# Autodesk Inventor assembly: Arm 2.0 Assembly
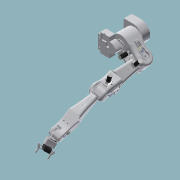
[picture p0: Inventor's stored thumbnail of the model, 180x180]
Saved by Autodesk Inventor 2017 SP1 (Build 210196100, 196)
## iProperties
Created: 2017-09-28
Part Number: Arm 2.0 Assembly
Document SubType Name: Assembly
Designer: Zach
Author: Zach
## Documents named in this file (66)
- C:\Users\Zach\Documents\GitHub\tr1\src\Body\Arm 2.0 Assembly\Arm 2.0 Assembly.iam
- C:\Users\Zach\Documents\GitHub\tr1\src\Body\Arm 2.0 Assembly\Steel Rod 8mm x 135mm.ipt
- C:\Users\Zach\Documents\GitHub\tr1\lib\22x8x8mm Bearing.ipt
- C:\Users\Zach\Documents\GitHub\tr1\src\Body\Arm 2.0 Assembly\AA004.ipt
- C:\Users\Zach\Documents\GitHub\tr1\lib\QS12MM250\QS12MM250.ipt
- C:\Users\Zach\Documents\GitHub\tr1\src\Body\Arm 2.0 Assembly\Steel Rod 8mm x 110mm.ipt
- C:\Users\Zach\Documents\GitHub\tr1\src\Body\Arm 2.0 Assembly\AA013.ipt
- C:\Users\Zach\Documents\GitHub\tr1\src\Body\Arm 2.0 Assembly\AA014.ipt
- C:\Users\Zach\Documents\GitHub\tr1\lib\12V DC Motor 378-1.ipt
- \\CR\Users\Zach\Documents\Inventor\Content Center Files\R2017\en-US\ISO 4017(1)\ISO 4017 - M5 x 20 - ISO.ipt
- C:\Users\Zach\Documents\GitHub\tr1\src\Body\Arm 2.0 Assembly\Steel Rod 8mm x 80mm.ipt
- C:\Users\Zach\Documents\GitHub\tr1\src\Body\Arm 2.0 Assembly\Gripper Assembly\Gripper B Assembly.iam
- C:\Users\Zach\Documents\GitHub\tr1\lib\8mm Hub.ipt
- C:\Users\Zach\Documents\GitHub\tr1\src\Body\Arm 2.0 Assembly\Arm 2.0 Assembly\Design Accelerator\Spur Gears5.iam
- C:\Users\Zach\Documents\GitHub\tr1\lib\4mm mounting hub.ipt
- C:\Users\Zach\Documents\GitHub\tr1\lib\6201RS\6201RS.ipt
- C:\Users\Zach\Documents\GitHub\tr1\lib\U51105\U51105.ipt
- C:\Users\Zach\Documents\GitHub\tr1\src\Body\Arm 2.0 Assembly\AA034.ipt
- C:\Users\Zach\Documents\GitHub\tr1\src\Body\Arm 2.0 Assembly\Arm 2.0 Assembly\Design Accelerator\Spur Gears6.iam
- C:\Users\Zach\Documents\GitHub\tr1\src\Body\Arm 2.0 Assembly\AA008c.ipt
- C:\Users\Zach\Documents\GitHub\tr1\src\Body\Arm 2.0 Assembly\Arm 2.0 Assembly\Design Accelerator\Spur Gears7.iam
- C:\Users\Zach\Documents\GitHub\tr1\src\Body\Arm 2.0 Assembly\AA036.ipt
- C:\Users\Zach\Documents\GitHub\tr1\src\Body\Arm 2.0 Assembly\AA037.ipt
- C:\Users\Zach\Documents\GitHub\tr1\src\Body\Arm 2.0 Assembly\AA016b.ipt
- C:\Users\Zach\Documents\GitHub\tr1\src\Body\Arm 2.0 Assembly\AA005b.ipt
- C:\Users\Zach\Documents\GitHub\tr1\src\Body\Arm 2.0 Assembly\AA006b.ipt
- C:\Users\Zach\Documents\GitHub\tr1\src\Body\Arm 2.0 Assembly\AA001c.ipt
- C:\Users\Zach\Documents\GitHub\tr1\src\Body\Arm 2.0 Assembly\Arm 2.0 Assembly\Design Accelerator\Spur Gears8.iam
- C:\Users\Zach\Documents\GitHub\tr1\src\Body\Arm 2.0 Assembly\Arm 2.0 Assembly\Design Accelerator\Spur Gears11.iam
- C:\Users\Zach\Documents\GitHub\tr1\src\Body\Arm 2.0 Assembly\Arm 2.0 Assembly\Design Accelerator\Spur Gears9.iam
- C:\Users\Zach\Documents\GitHub\tr1\src\Body\Arm 2.0 Assembly\AA010b.ipt
- C:\Users\Zach\Documents\GitHub\tr1\src\Body\Arm 2.0 Assembly\Arm 2.0 Assembly\Design Accelerator\Spur Gears10.iam
- C:\Users\Zach\Documents\GitHub\tr1\src\Body\Arm 2.0 Assembly\Arm 2.0 Assembly\Design Accelerator\Spur Gears12.iam
- C:\Users\Zach\Documents\GitHub\tr1\src\Body\Arm 2.0 Assembly\AA041.ipt
- \\CR\Users\Zach\Documents\Inventor\Content Center Files\R2017\en-US\ISO 7045  H\ISO 7045 - M3 x 8 - 4.8 - H - ISO.ipt
- C:\Users\Zach\Documents\GitHub\tr1\src\Body\Arm 2.0 Assembly\Arm 2.0 Assembly\Design Accelerator\Spur Gears13.iam
- C:\Users\Zach\Documents\GitHub\tr1\src\Body\Arm 2.0 Assembly\Arm 2.0 Assembly\Design Accelerator\Spur Gears16.iam
- C:\Users\Zach\Documents\GitHub\tr1\src\Body\Arm 2.0 Assembly\AA046.ipt
- C:\Users\Zach\Documents\GitHub\tr1\lib\MG995.ipt
- C:\Users\Zach\Documents\GitHub\tr1\lib\Servo Mounting Hub.ipt
- C:\Users\Zach\Documents\GitHub\tr1\src\Body\Arm 2.0 Assembly\AA047.ipt
- C:\Users\Zach\Documents\GitHub\tr1\src\Body\Arm 2.0 Assembly\AA048.ipt
- \\CR\Users\Zach\Documents\Inventor\Content Center Files\R2017\en-US\ISO 4018\ISO 4018 - M5 x 10.ipt
- \\CR\Users\Zach\Documents\Inventor\Content Center Files\R2017\en-US\ISO 4018\ISO 4018 - M5 x 25.ipt
- \\CR\Users\Zach\Documents\Inventor\Content Center Files\R2017\en-US\ISO 7045  H\ISO 7045 - M3 x 12 - 4.8 - H - ISO.ipt
- C:\Users\Zach\Documents\GitHub\tr1\src\Body\Arm 2.0 Assembly\AA049.ipt
- \\CR\Users\Zach\Documents\Inventor\Content Center Files\R2017\en-US\ISO 4018\ISO 4018 - M5 x 40.ipt
- \\CR\Users\Zach\Documents\Inventor\Content Center Files\R2017\en-US\ISO 4035(2)\ISO 4035 - M5 - ISO.ipt
- \\CR\Users\Zach\Documents\Inventor\Content Center Files\R2017\en-US\ISO 4018\ISO 4018 - M5 x 35.ipt
- \\CR\Users\Zach\Documents\Inventor\Content Center Files\R2017\en-US\ISO 4762(2)\ISO 4762 - M4 x 10ISO.ipt
- C:\Users\Zach\Documents\GitHub\tr1\lib\6mm Mounting Hub.ipt
- C:\Users\Zach\Documents\GitHub\tr1\src\Body\Arm 2.0 Assembly\AA035c.ipt
- C:\Users\Zach\Documents\GitHub\tr1\src\Body\Arm 2.0 Assembly\AA008d2.ipt
- C:\Users\Zach\Documents\GitHub\tr1\lib\TSINY TS-42GZ495.ipt
- C:\Users\Zach\Documents\GitHub\tr1\lib\EMS22XXX-D28-LSX.ipt
- C:\Users\Zach\Documents\GitHub\tr1\src\Body\Arm 2.0 Assembly\AA051.ipt
- C:\Users\Zach\Documents\GitHub\tr1\src\Body\Arm 2.0 Assembly\AA052.ipt
- C:\Users\Zach\Documents\GitHub\tr1\src\Body\Arm 2.0 Assembly\AA045b.ipt
- C:\Users\Zach\Documents\GitHub\tr1\lib\6mm x 120mm D Shaft.ipt
- C:\Users\Zach\Documents\GitHub\tr1\src\Body\Arm 2.0 Assembly\AA053.ipt
- C:\Users\Zach\Documents\GitHub\tr1\src\Body\Arm 2.0 Assembly\AA054.ipt
- C:\Users\Zach\Documents\GitHub\tr1\src\Body\Arm 2.0 Assembly\AA055.ipt
- \\CR\Users\Zach\Documents\Inventor\Content Center Files\R2017\en-US\AS 1421(4)\AS 1421 - M4 x 10 Flat Point.ipt
- C:\Users\Zach\Documents\GitHub\tr1\src\Body\Arm 2.0 Assembly\AA057.ipt
- C:\Users\Zach\Documents\GitHub\tr1\lib\6mm Mounting Hub, thin.ipt
- C:\Users\Zach\Documents\GitHub\tr1\lib\8mm Mounting Hub, thin.ipt
## Components (202 placed, 65 different names)
1. AA001c:1 — Mate:560, Mate:562, Mate:563, Mate:564, Mate:565, Mate:566, Mate:567, Mate:576, Mate:578, Mate:581, Mate:602, Mate:905, Mate:906, Mate:1083, Mate:1084, Mate:1085, Mate:1086, Mate:1093, Angle:18, Mate:1095, Mate:1122, Mate:1261, Mate:1262, Mate:1263, Mate:1278, Mate:1279, Mate:1280, Mate:1294
2. AA004:1 — Mate:23, Mate:345, Mate:347, Mate:350, Mate:357, Mate:590, Mate:1278
3. AA005b:1 — Mate:537, Mate:538, Mate:539, Mate:541, Mate:542, Mate:543, Mate:806, Mate:807, Mate:808, Mate:809, Mate:838, Mate:909, Mate:910
4. AA006b:1 — Mate:594, Mate:598, Mate:599, Mate:609, Mate:802, Mate:803, Mate:804, Mate:805, Mate:838, Mate:1088, Mate:1089, Angle:17, Mate:1233
5. AA008c:1 — Mate:616, Mate:1113, Mate:1114, Mate:1115, Mate:1125
6. AA008d2:1 — Mate:1104, Mate:1106, Mate:1107, Angle:22, Mate:1113, Mate:1114, Mate:1115, Mate:1124, Mate:1125, Mate:1157, Mate:1158, Mate:1159, Mate:1160, Mate:1161, Mate:1162, Mate:1163, Mate:1164, Mate:1165, Mate:1166, Mate:1170, Mate:1192, Mate:1193, Mate:1194, Mate:1195, Mate:1312
7. AA010b:1 — Mate:616, Mate:620, Mate:621, Mate:624, Mate:625, Mate:626, Mate:628, Mate:630, Mate:642, Flush:20, Mate:648, Mate:650, Mate:948, Mate:1097, Mate:1098, Angle:21, Mate:1100, Mate:1101, Mate:1102, Mate:1126, Mate:1204, Mate:1258, Mate:1259, Mate:1260, Mate:1274, Mate:1276, Mate:1277, Mate:1301
8. AA013:2 — Mate:142, Mate:143, Mate:144, Mate:145, Mate:146, Mate:147, Mate:563, Mate:564, Mate:565, Mate:1281
9. AA014:2 — Mate:628, Mate:629, Mate:630, Mate:976, Mate:977, Mate:978, Mate:979, Mate:980, Mate:981
10. AA016b:1 — Mate:518, Mate:519, Mate:520, Mate:529, Mate:530, Mate:664, Mate:665, Mate:671, Mate:673, Mate:675, Mate:676, Mate:677, Mate:877, Mate:878, Mate:1206, Mate:1207, Angle:26
11. AA034:1 — Mate:529, Mate:534, Mate:535, Mate:879, Mate:880, Mate:881, Mate:882, Mate:883, Mate:884, Mate:885, Mate:886, Mate:964, Mate:965, Mate:966, Mate:967, Mate:968, Mate:969, Mate:970, Mate:971, Mate:972, Mate:973, Mate:974, Mate:975, Mate:1213, Mate:1256, Mate:1309, Mate:1310, Mate:1311
12. AA035c:1 — Mate:1076, Mate:1077, Mate:1167, Mate:1168, Mate:1169, Mate:1170, Mate:1171, Mate:1172, Mate:1173, Mate:1175, Angle:24, Angle:25, Mate:1176, Mate:1202, Mate:1203, Angle:1297, Mate:1312
13. AA036:1 — Mate:498, Mate:501, Mate:502, Mate:511, Mate:698, Mate:868, Mate:871, Mate:872, Mate:939, Mate:1197, Mate:1198, Mate:1199, Mate:1200
14. AA037:1 — Mate:501, Mate:502, Mate:514, Mate:515, Mate:516, Mate:518, Mate:519, Mate:520, Mate:530, Mate:664, Mate:665, Mate:698, Mate:866, Mate:867, Mate:873, Mate:874, Mate:875, Mate:876, Flush:25, Flush:26, Mate:950, Mate:951, Mate:952, Mate:953
15. AA041:1 — Mate:675, Mate:676, Mate:677, Mate:682, Mate:683, Mate:684, Mate:685
16. AA045b:1 — Mate:1211, Mate:1212, Angle:27, Mate:1213, Mate:1214, Mate:1215, Mate:1216, Mate:1217, Mate:1218, Mate:1219, Flush:37, Mate:1221, Mate:1223, Mate:1224, Mate:1225, Mate:1227, Mate:1235, Mate:1264, Mate:1265, Mate:1310, Mate:1311
17. AA046:1 — Mate:727, Mate:728, Mate:731, Mate:735, Mate:736, Mate:737, Mate:752, Mate:756, Mate:758, Mate:759, Mate:760, Mate:761, Mate:762, Mate:763, Mate:1217, Mate:1296, Mate:1297
18. AA047:1 — Mate:735, Mate:736, Mate:737, Mate:738, Mate:739, Mate:740, Mate:753, Mate:754, Mate:755, Mate:800, Mate:801
19. AA048:1 — Mate:744, Mate:745, Mate:746, Mate:747, Mate:748, Mate:749
20. AA049:1 — Mate:783, Mate:786, Mate:787, Mate:788, Mate:789, Mate:790, Mate:791, Mate:1218
21. AA051:1 — Mate:1196, Mate:1197
22. AA052:1 — Mate:1201, Mate:1202
23. AA053:1 — Mate:1258, Mate:1259, Mate:1260
24. AA053:3 — Mate:1261, Mate:1262, Mate:1263
25. AA054:1 — Mate:1270, Mate:1271, Mate:1275, Mate:1276, Mate:1282, Mate:1320
26. AA055:1 — Mate:1274, Mate:1275, Mate:1277
27. AA057:1 — Mate:1293, Angle:1295, Mate:1294, Mate:1295
28. AA057:2 — Mate:1300, Angle:1296, Mate:1301, Mate:1302
29. Gripper B Assembly:1 [sub-assembly] — Mate:747, Mate:748, Mate:749
30. 22x8x8mm Bearing:1 — Mate:433, Mate:560
31. 22x8x8mm Bearing:2 — Mate:437, Mate:562
32. 22x8x8mm Bearing:3 — Mate:57, Mate:620, Mate:626
33. 22x8x8mm Bearing:4 — Mate:621, Mate:629, Mate:642
34. 22x8x8mm Bearing:5 — Mate:186, Mate:1265
35. 22x8x8mm Bearing:6 — Mate:187, Mate:1264
36. 22x8x8mm Bearing:7 — Mate:1308
37. QS12MM250:1 — Mate:23, Mate:344, Mate:346, Mate:348, Mate:354, Mate:537, Mate:594, Mate:597, Mate:1230
38. Steel Rod 8mm x 140mm:1 — Mate:433, Mate:437, Mate:476, Mate:575, Mate:651, Mate:1076, Mate:1122, Flush:35, Mate:1201
39. Steel Rod 8mm x 110mm:1 — Mate:57, Mate:491, Mate:498, Flush:20, Mate:649, Mate:1196, Mate:1204, Mate:1283
40. Steel Rod 8mm x 80mm:1 — Mate:186, Mate:187, Mate:710, Mate:721, Mate:724, Mate:730, Mate:783, Mate:1216, Flush:37, Mate:1234, Mate:1298, Mate:1299
41. TSINY TS-42GZ495:3 — Mate:1104, Mate:1160, Mate:1161, Mate:1270, Mate:1271, Angle:1297
42. TSINY TS-42GZ495:2 — Mate:1097, Mate:1098, Mate:1101, Mate:1102, Mate:1128, Mate:1300, Angle:1296
43. TSINY TS-42GZ495:1 — Mate:1083, Mate:1084, Mate:1085, Mate:1086, Mate:1293, Angle:1295
44. 12V DC Motor 378-1:3 — Mate:712, Mate:714, Mate:778, Mate:779, Mate:1224, Mate:1225
45. 12V DC Motor 378-1:4 — Mate:514, Mate:515, Mate:516, Mate:1290, Mate:1292, Mate:1303, Mate:1304
46. 12V DC Motor 378-1:6 — Mate:340, Mate:342, Mate:538, Mate:539, Mate:540, Mate:543, Mate:907, Mate:908
47. 6201RS:1 — Mate:346, Mate:347
48. 6201RS:2 — Mate:357, Mate:597
49. U51105:1 — Mate:348, Mate:349, Mate:542
50. U51105:2 — Mate:354, Mate:608, Mate:609, Mate:600
51. 6mm Mounting Hub:7 — Mate:1185, Mate:1186, Mate:1188
52. 6mm Mounting Hub:5 — Mate:1177, Mate:1178, Mate:1179
53. 6mm Mounting Hub:2 — Mate:1090, Mate:1091
54. 6mm Mounting Hub:11 — Mate:1283, Mate:1284
55. 6mm Mounting Hub:10 — Mate:1228, Mate:1323
56. 8mm Hub:2 — Mate:534, Mate:535, Mate:1306
57. 8mm Hub:4 — Mate:580, Mate:581, Mate:582, Flush:35
58. 8mm Hub:6 — Mate:651, Mate:911, Mate:912, Mate:913, Mate:914, Mate:915, Mate:916, Mate:1203
59. 8mm Hub:8 — Mate:721, Mate:1234, Mate:1324, Mate:1325
60. 8mm Hub:9 — Mate:727, Mate:728, Mate:730, Mate:756, Mate:764, Mate:765, Mate:766, Mate:767, Mate:768, Mate:769, Mate:1298, Mate:1299
61. 8mm Hub:14 — Mate:1198, Mate:1199, Mate:1200
62. 4mm mounting hub:1 — Mate:340, Mate:540, Mate:541, Mate:887
63. 4mm mounting hub:8 — Mate:714, Mate:716, Mate:782, Mate:1226
64. Servo Mounting Hub:1 — Mate:733, Mate:734, Mate:738, Mate:739, Mate:740, Mate:792, Mate:793, Mate:794, Mate:795, Mate:796, Mate:797, Mate:798, Mate:799
65. 6mm x 120mm D Shaft:1 — Mate:1292, Mate:1303, Mate:1304, Mate:1305, Mate:1306, Mate:1308, Mate:1309, Mate:1318
66. EMS22XXX-D28-LSX:1 — Mate:1088, Mate:1089, Angle:17, Mate:1090, Mate:1091, Mate:1182, Mate:1232
67. EMS22XXX-D28-LSX:2 — Mate:1093, Angle:18, Mate:1095, Mate:1177, Mate:1180
68. EMS22XXX-D28-LSX:3 — Angle:21, Mate:1100, Mate:1126, Mate:1185, Mate:1187
69. EMS22XXX-D28-LSX:4 — Mate:1106, Mate:1107, Angle:22, Mate:1190, Mate:1313
70. EMS22XXX-D28-LSX:5 — Mate:1206, Mate:1207, Angle:26, Mate:1210, Mate:1316, Mate:1326
71. EMS22XXX-D28-LSX:6 — Mate:1211, Mate:1212, Angle:27, Mate:1228, Mate:1267
72. AASG01 [sub-assembly] — Mate:342, Mate:344, Mate:345, Mate:349, Mate:350, Mate:810, Mate:811, Mate:812, Mate:813, Mate:814, Mate:815, Mate:816, Mate:817, Mate:818, Mate:819, Mate:820, Mate:821, Mate:887, Mate:888, Mate:889, Mate:890, Mate:891, Mate:1279, Mate:1280
73. AASG02 [sub-assembly] — Mate:476, Mate:566, Mate:567, Mate:602, Mate:839, Mate:841, Mate:842, Mate:843, Mate:844, Mate:845, Mate:897, Mate:898, Mate:899, Mate:900, Mate:901, Mate:902, Mate:1077, Mate:1295
74. AASG03 [sub-assembly] — Mate:491, Mate:511, Mate:624, Mate:625, Mate:860, Mate:861, Mate:862, Mate:863, Mate:864, Mate:865, Mate:1128, Mate:1302
75. AASG04 [sub-assembly] — Mate:575, Mate:576, Mate:578, Mate:580, Mate:582, Mate:917, Mate:918, Mate:919, Mate:920, Mate:921, Mate:922, Mate:1178, Mate:1179, Mate:1180
76. AASG05 [sub-assembly] — Mate:590, Mate:608, Mate:827, Mate:828, Mate:829, Mate:830, Mate:831, Mate:832, Mate:833, Mate:1182, Mate:1230, Mate:1232, Mate:1233
77. AASG06 [sub-assembly] — Mate:1124, Mate:1190, Mate:1268, Mate:1269, Mate:1282, Mate:1314, Mate:1315, Mate:1321, Mate:1322
78. AASG07 [sub-assembly] — Mate:648, Mate:649, Mate:650, Mate:958, Mate:959, Mate:960, Mate:961, Mate:962, Mate:963, Mate:1186, Mate:1187, Mate:1188, Mate:1284
79. AASG08 [sub-assembly] — Mate:671, Mate:673, Mate:680, Mate:681, Mate:1305, Mate:1317, Mate:1319, Mate:1326
80. AASG09 [sub-assembly] — Mate:710, Mate:712, Mate:716, Mate:731, Mate:770, Mate:771, Mate:772, Mate:773, Mate:774, Mate:775, Mate:776, Mate:777, Mate:782, Mate:1223, Mate:1226, Mate:1227, Mate:1296, Mate:1297
81. AASG10 [sub-assembly] — Mate:724, Mate:1221, Mate:1235, Mate:1267, Mate:1323, Mate:1324, Mate:1325
82. MG995:1 — Mate:733, Mate:734, Mate:744, Mate:745, Mate:746
83. 6mm Mounting Hub, thin:1 — Mate:1313, Mate:1314, Mate:1315
84. ISO 7045 H M3 x 8 - 4.8 - H:1 — Mate:680, Mate:681
85. ISO 7045 H M3 x 8 - 4.8 - H:2 — Mate:682, Mate:685
86. ISO 7045 H M3 x 8 - 4.8 - H:3 — Mate:683, Mate:684
87. ISO 7045 H M3 x 8 - 4.8 - H:5 — Mate:778
88. ISO 7045 H M3 x 8 - 4.8 - H:6 — Mate:779
89. ISO 7045 H M3 x 8 - 4.8 - H:7 — Mate:795, Mate:799
90. ISO 7045 H M3 x 8 - 4.8 - H:8 — Mate:794, Mate:798
91. ISO 7045 H M3 x 8 - 4.8 - H:9 — Mate:792, Mate:796
92. ISO 7045 H M3 x 8 - 4.8 - H:10 — Mate:793, Mate:797
93. ISO 7045 H M3 x 8 - 4.8 - H:11 — Mate:800, Mate:801
94. ISO 7045 H M3 x 8 - 4.8 - H:13 — Mate:897, Mate:900
95. ISO 7045 H M3 x 8 - 4.8 - H:14 — Mate:898, Mate:901
96. ISO 7045 H M3 x 8 - 4.8 - H:15 — Mate:899, Mate:902
97. ISO 7045 H M3 x 8 - 4.8 - H:16 — Mate:908, Mate:910
98. ISO 7045 H M3 x 8 - 4.8 - H:17 — Mate:907, Mate:909
99. ISO 7045 H M3 x 8 - 4.8 - H:20 — Mate:951, Mate:953
100. ISO 7045 H M3 x 8 - 4.8 - H:21 — Mate:950, Mate:952
101. ISO 7045 H M3 x 8 - 4.8 - H:24 — Mate:960, Mate:963
102. ISO 7045 H M3 x 8 - 4.8 - H:25 — Mate:958, Mate:962
103. ISO 7045 H M3 x 8 - 4.8 - H:26 — Mate:959, Mate:961
104. ISO 7045 H M3 x 8 - 4.8 - H:27 — Mate:965, Mate:972
105. ISO 7045 H M3 x 8 - 4.8 - H:28 — Mate:964, Mate:973
106. ISO 7045 H M3 x 8 - 4.8 - H:29 — Mate:966, Mate:971
107. ISO 7045 H M3 x 8 - 4.8 - H:30 — Mate:967, Mate:970, Mate:1256
108. ISO 7045 H M3 x 8 - 4.8 - H:31 — Mate:969, Mate:975
109. ISO 7045 H M3 x 8 - 4.8 - H:32 — Mate:968, Mate:974
110. ISO 7045 H M3 x 12 - 4.8 - H:1 — Mate:765, Mate:767
111. ISO 7045 H M3 x 12 - 4.8 - H:3 — Mate:764, Mate:769
112. ISO 7045 H M3 x 12 - 4.8 - H:2 — Mate:766, Mate:768
113. ISO 7045 H M3 x 12 - 4.8 - H:4 — Mate:770, Mate:775
114. ISO 7045 H M3 x 12 - 4.8 - H:5 — Mate:771, Mate:774
115. ISO 7045 H M3 x 12 - 4.8 - H:6 — Mate:773, Mate:777
116. ISO 7045 H M3 x 12 - 4.8 - H:7 — Mate:772, Mate:776
117. ISO 7045 H M3 x 12 - 4.8 - H:8 — Mate:889, Mate:890
118. ISO 7045 H M3 x 12 - 4.8 - H:9 — Mate:888, Mate:891
119. ISO 7045 H M3 x 12 - 4.8 - H:10 — Mate:911, Mate:914
120. ISO 7045 H M3 x 12 - 4.8 - H:11 — Mate:913, Mate:915
121. ISO 7045 H M3 x 12 - 4.8 - H:12 — Mate:912, Mate:916
122. ISO 7045 H M3 x 12 - 4.8 - H:13 — Mate:919, Mate:920
123. ISO 7045 H M3 x 12 - 4.8 - H:14 — Mate:917, Mate:921
124. ISO 7045 H M3 x 12 - 4.8 - H:15 — Mate:918, Mate:922
125. ISO 7045 H M3 x 12 - 4.8 - H:18
126. ISO 7045 H M3 x 12 - 4.8 - H:19
127. ISO 7045 H M3 x 12 - 4.8 - H:20
128. ISO 7045 H M3 x 12 - 4.8 - H:32 — Mate:1268, Mate:1269
129. ISO 4762 M4 x 10:1 — Mate:905
130. ISO 4762 M4 x 10:2 — Mate:906
131. ISO 4762 M4 x 10:4 — Mate:948
132. ISO 4035 M5:1 — Mate:1167, Mate:1168
133. ISO 4035 M5:2 — Mate:852, Mate:1176
134. ISO 4035 M5:3 — Mate:869, Mate:872
135. ISO 4035 M5:4 — Mate:870, Mate:871
136. ISO 4035 M5:5 — Mate:985
137. ISO 4035 M5:6 — Mate:984
138. ISO 4035 M5:7 — Mate:989
139. ISO 4035 M5:8 — Mate:988
140. ISO 4035 M5:9 — Mate:1174, Mate:1175, Angle:24
141. ISO 4035 M5:10 — Mate:1027, Mate:1173, Angle:25
142. ISO 4018 M5 x 10:1 — Mate:754, Mate:755
143. ISO 4018 M5 x 10:2 — Mate:752, Mate:753
144. ISO 4018 M5 x 10:3 — Mate:787, Mate:790
145. ISO 4018 M5 x 10:4 — Mate:788, Mate:791
146. ISO 4018 M5 x 10:5 — Mate:786, Mate:789, Mate:1219
147. ISO 4017 M5 x 20:1 — Mate:146, Mate:147, Mate:1281
148. ISO 4017 M5 x 20:2 — Mate:144, Mate:145
149. ISO 4017 M5 x 20:3 — Mate:142, Mate:143
150. ISO 4017 M5 x 20:4 — Mate:978, Mate:980
151. ISO 4017 M5 x 20:5 — Mate:977, Mate:979
152. ISO 4017 M5 x 20:6 — Mate:976, Mate:981
153. ISO 4018 M5 x 25:1 — Mate:758, Mate:761
154. ISO 4018 M5 x 25:2 — Mate:759, Mate:763
155. ISO 4018 M5 x 25:3 — Mate:760, Mate:762
156. ISO 4018 M5 x 25:7 — Mate:802, Mate:803
157. ISO 4018 M5 x 25:8 — Mate:804, Mate:805
158. ISO 4018 M5 x 25:9 — Mate:806, Mate:808
159. ISO 4018 M5 x 25:10 — Mate:807, Mate:809
160. ISO 4018 M5 x 25:11 — Mate:812, Mate:820
161. ISO 4018 M5 x 25:12 — Mate:810, Mate:816
162. ISO 4018 M5 x 25:13 — Mate:811, Mate:821
163. ISO 4018 M5 x 25:14 — Mate:814, Mate:817
164. ISO 4018 M5 x 25:15 — Mate:813, Mate:819
165. ISO 4018 M5 x 25:16 — Mate:815, Mate:818
166. ISO 4018 M5 x 25:17 — Mate:831
167. ISO 4018 M5 x 25:18 — Mate:829
168. ISO 4018 M5 x 25:19 — Mate:832
169. ISO 4018 M5 x 25:20 — Mate:827, Mate:828
170. ISO 4018 M5 x 25:21 — Mate:833
171. ISO 4018 M5 x 25:22 — Mate:830
172. ISO 4018 M5 x 25:23
173. ISO 4018 M5 x 25:24
174. ISO 4018 M5 x 25:25 — Mate:839, Mate:845
175. ISO 4018 M5 x 25:27 — Mate:841, Mate:844
176. ISO 4018 M5 x 25:28 — Mate:842, Mate:843
177. ISO 4018 M5 x 25:29 — Mate:1157, Mate:1159
178. ISO 4018 M5 x 25:30 — Mate:1192, Mate:1193
179. ISO 4018 M5 x 25:31 — Mate:1194, Mate:1195
180. ISO 4018 M5 x 25:32 — Mate:1158
181. ISO 4018 M5 x 25:33 — Mate:860, Mate:865, Mate:939
182. ISO 4018 M5 x 25:34 — Mate:862, Mate:863
183. ISO 4018 M5 x 25:35 — Mate:861, Mate:864
184. ISO 4018 M5 x 25:36 — Mate:876, Mate:878
185. ISO 4018 M5 x 25:37 — Mate:875, Mate:877
186. ISO 4018 M5 x 25:38 — Mate:874, Flush:26
187. ISO 4018 M5 x 25:39 — Mate:873, Flush:25
188. ISO 4018 M5 x 25:40 — Mate:882, Mate:883, Mate:984
189. ISO 4018 M5 x 25:41 — Mate:880, Mate:886, Mate:988, Mate:1214
190. ISO 4018 M5 x 25:42 — Mate:879, Mate:885, Mate:985
191. ISO 4018 M5 x 25:43 — Mate:881, Mate:884, Mate:989, Mate:1215
192. ISO 4018 M5 x 35:1 — Mate:866, Mate:867, Flush:24, Mate:869
193. ISO 4018 M5 x 35:2 — Mate:868, Flush:24, Mate:870
194. ISO 4018 M5 x 40:1 — Mate:1162, Mate:1169
195. ISO 4018 M5 x 40:2 — Mate:852, Mate:1163, Mate:1166
196. ISO 4018 M5 x 40:3 — Mate:1027, Mate:1165, Mate:1172
197. ISO 4018 M5 x 40:4 — Mate:1164, Mate:1171, Mate:1174
198. AS 1421 Flat Point - Metric M4 x 10 Flat Point:1
199. AS 1421 Flat Point - Metric M4 x 10 Flat Point:2 — Mate:1290
200. 6mm Mounting Hub, thin:2 — Mate:1316, Mate:1317, Mate:1210
201. 6mm Mounting Hub, thin:3 — Mate:1318, Mate:1319
202. 8mm Mounting Hub, thin:1 — Mate:1320, Mate:1321, Mate:1322
## Relationships (463: Mate 446, Angle 11, Flush 6)
- Mate:23: AA004:1 ↔ QS12MM250:1
- Mate:57: 22x8x8mm Bearing:3 ↔ Steel Rod 8mm x 110mm:1
- Mate:142: AA013:2 ↔ ISO 4017 M5 x 20:3
- Mate:143: AA013:2 ↔ ISO 4017 M5 x 20:3
- Mate:144: AA013:2 ↔ ISO 4017 M5 x 20:2
- Mate:145: AA013:2 ↔ ISO 4017 M5 x 20:2
- Mate:146: AA013:2 ↔ ISO 4017 M5 x 20:1
- Mate:147: AA013:2 ↔ ISO 4017 M5 x 20:1
- Mate:186: 22x8x8mm Bearing:5 ↔ Steel Rod 8mm x 80mm:1
- Mate:187: 22x8x8mm Bearing:6 ↔ Steel Rod 8mm x 80mm:1
- Mate:340: 12V DC Motor 378-1:6 ↔ 4mm mounting hub:1
- Mate:342: 12V DC Motor 378-1:6 ↔ AASG01
- Mate:344: QS12MM250:1 ↔ AASG01
- Mate:345: AA004:1 ↔ AASG01
- Mate:346: QS12MM250:1 ↔ 6201RS:1
- Mate:347: AA004:1 ↔ 6201RS:1
- Mate:348: QS12MM250:1 ↔ U51105:1
- Mate:349: U51105:1 ↔ AASG01
- Mate:350: AA004:1 ↔ AASG01
- Mate:354: QS12MM250:1 ↔ U51105:2
- Mate:357: AA004:1 ↔ 6201RS:2
- Mate:433: 22x8x8mm Bearing:1 ↔ Steel Rod 8mm x 140mm:1
- Mate:437: 22x8x8mm Bearing:2 ↔ Steel Rod 8mm x 140mm:1
- Mate:476: Steel Rod 8mm x 140mm:1 ↔ AASG02
- Mate:491: Steel Rod 8mm x 110mm:1 ↔ AASG03
- Mate:498: AA036:1 ↔ Steel Rod 8mm x 110mm:1
- Mate:501: AA036:1 ↔ AA037:1
- Mate:502: AA036:1 ↔ AA037:1
- Mate:511: AA036:1 ↔ AASG03
- Mate:514: AA037:1 ↔ 12V DC Motor 378-1:4
- Mate:515: AA037:1 ↔ 12V DC Motor 378-1:4
- Mate:516: AA037:1 ↔ 12V DC Motor 378-1:4
- Mate:518: AA016b:1 ↔ AA037:1
- Mate:519: AA016b:1 ↔ AA037:1
- Mate:520: AA016b:1 ↔ AA037:1
- Mate:529: AA016b:1 ↔ AA034:1
- Mate:530: AA016b:1 ↔ AA037:1
- Mate:534: AA034:1 ↔ 8mm Hub:2
- Mate:535: AA034:1 ↔ 8mm Hub:2
- Mate:537: AA005b:1 ↔ QS12MM250:1
- Mate:538: AA005b:1 ↔ 12V DC Motor 378-1:6
- Mate:539: AA005b:1 ↔ 12V DC Motor 378-1:6
- Mate:540: 12V DC Motor 378-1:6 ↔ 4mm mounting hub:1
- Mate:541: AA005b:1 ↔ 4mm mounting hub:1
- Mate:542: AA005b:1 ↔ U51105:1
- Mate:543: AA005b:1 ↔ 12V DC Motor 378-1:6
- Mate:560: AA001c:1 ↔ 22x8x8mm Bearing:1
- Mate:562: AA001c:1 ↔ 22x8x8mm Bearing:2
- Mate:563: AA001c:1 ↔ AA013:2
- Mate:564: AA001c:1 ↔ AA013:2
- Mate:565: AA001c:1 ↔ AA013:2
- Mate:566: AA001c:1 ↔ AASG02
- Mate:567 (1 mm): AA001c:1 ↔ AASG02
- Mate:575: Steel Rod 8mm x 140mm:1 ↔ AASG04
- Mate:576: AA001c:1 ↔ AASG04
- Mate:578: AA001c:1 ↔ AASG04
- Mate:580: 8mm Hub:4 ↔ AASG04
- Mate:581: AA001c:1 ↔ 8mm Hub:4
- Mate:582: 8mm Hub:4 ↔ AASG04
- Mate:590: AA004:1 ↔ AASG05
- Mate:594: AA006b:1 ↔ QS12MM250:1
- Mate:597: QS12MM250:1 ↔ 6201RS:2
- Mate:598: AA006b:1
- Mate:599: AA006b:1
- Mate:600: U51105:2
- Mate:602 (2.5 mm): AA001c:1 ↔ AASG02
- Mate:608: U51105:2 ↔ AASG05
- Mate:609: AA006b:1 ↔ U51105:2
- Mate:616: AA008c:1 ↔ AA010b:1
- Mate:620: AA010b:1 ↔ 22x8x8mm Bearing:3
- Mate:621: AA010b:1 ↔ 22x8x8mm Bearing:4
- Mate:624: AA010b:1 ↔ AASG03
- Mate:625: AA010b:1 ↔ AASG03
- Flush:20 (0.5 mm): AA010b:1 ↔ Steel Rod 8mm x 110mm:1
- Mate:626: AA010b:1 ↔ 22x8x8mm Bearing:3
- Mate:628: AA010b:1 ↔ AA014:2
- Mate:629: AA014:2 ↔ 22x8x8mm Bearing:4
- Mate:630: AA010b:1 ↔ AA014:2
- Mate:642: AA010b:1 ↔ 22x8x8mm Bearing:4
- Mate:648: AA010b:1 ↔ AASG07
- Mate:649: Steel Rod 8mm x 110mm:1 ↔ AASG07
- Mate:650: AA010b:1 ↔ AASG07
- Mate:651: Steel Rod 8mm x 140mm:1 ↔ 8mm Hub:6
- Mate:664: AA016b:1 ↔ AA037:1
- Mate:665: AA016b:1 ↔ AA037:1
- Mate:671: AA016b:1 ↔ AASG08
- Mate:673: AA016b:1 ↔ AASG08
- Mate:675: AA016b:1 ↔ AA041:1
- Mate:676: AA016b:1 ↔ AA041:1
- Mate:677: AA016b:1 ↔ AA041:1
- Mate:680: AASG08 ↔ ISO 7045 H M3 x 8 - 4.8 - H:1
- Mate:681: AASG08 ↔ ISO 7045 H M3 x 8 - 4.8 - H:1
- Mate:682: AA041:1 ↔ ISO 7045 H M3 x 8 - 4.8 - H:2
- Mate:683: AA041:1 ↔ ISO 7045 H M3 x 8 - 4.8 - H:3
- Mate:684: AA041:1 ↔ ISO 7045 H M3 x 8 - 4.8 - H:3
- Mate:685: AA041:1 ↔ ISO 7045 H M3 x 8 - 4.8 - H:2
- Mate:698: AA036:1 ↔ AA037:1
- Mate:710: Steel Rod 8mm x 80mm:1 ↔ AASG09
- Mate:712: 12V DC Motor 378-1:3 ↔ AASG09
- Mate:714: 12V DC Motor 378-1:3 ↔ 4mm mounting hub:8
- Mate:716: 4mm mounting hub:8 ↔ AASG09
- Mate:721: Steel Rod 8mm x 80mm:1 ↔ 8mm Hub:8
- Mate:724: Steel Rod 8mm x 80mm:1 ↔ AASG10
- Mate:727: AA046:1 ↔ 8mm Hub:9
- Mate:728: AA046:1 ↔ 8mm Hub:9
- Mate:730: Steel Rod 8mm x 80mm:1 ↔ 8mm Hub:9
- Mate:731: AA046:1 ↔ AASG09
- Mate:733: Servo Mounting Hub:1 ↔ MG995:1
- Mate:734: Servo Mounting Hub:1 ↔ MG995:1
- Mate:735: AA046:1 ↔ AA047:1
- Mate:736: AA046:1 ↔ AA047:1
- Mate:737: AA046:1 ↔ AA047:1
- Mate:738: AA047:1 ↔ Servo Mounting Hub:1
- Mate:739: AA047:1 ↔ Servo Mounting Hub:1
- Mate:740: AA047:1 ↔ Servo Mounting Hub:1
- Mate:744: AA048:1 ↔ MG995:1
- Mate:745 (0.5 mm): AA048:1 ↔ MG995:1
- Mate:746 (0.5 mm): AA048:1 ↔ MG995:1
- Mate:747: AA048:1 ↔ Gripper B Assembly:1
- Mate:748: AA048:1 ↔ Gripper B Assembly:1
- Mate:749: AA048:1 ↔ Gripper B Assembly:1
- Mate:752: AA046:1 ↔ ISO 4018 M5 x 10:2
- Mate:753: AA047:1 ↔ ISO 4018 M5 x 10:2
- Mate:754: AA047:1 ↔ ISO 4018 M5 x 10:1
- Mate:755: AA047:1 ↔ ISO 4018 M5 x 10:1
- Mate:756: AA046:1 ↔ 8mm Hub:9
- Mate:758: AA046:1 ↔ ISO 4018 M5 x 25:1
- Mate:759: AA046:1 ↔ ISO 4018 M5 x 25:2
- Mate:760: AA046:1 ↔ ISO 4018 M5 x 25:3
- Mate:761: AA046:1 ↔ ISO 4018 M5 x 25:1
- Mate:762: AA046:1 ↔ ISO 4018 M5 x 25:3
- Mate:763: AA046:1 ↔ ISO 4018 M5 x 25:2
- Mate:764: 8mm Hub:9 ↔ ISO 7045 H M3 x 12 - 4.8 - H:3
- Mate:765: 8mm Hub:9 ↔ ISO 7045 H M3 x 12 - 4.8 - H:1
- Mate:766: 8mm Hub:9 ↔ ISO 7045 H M3 x 12 - 4.8 - H:2
- Mate:767: 8mm Hub:9 ↔ ISO 7045 H M3 x 12 - 4.8 - H:1
- Mate:768: 8mm Hub:9 ↔ ISO 7045 H M3 x 12 - 4.8 - H:2
- Mate:769: 8mm Hub:9 ↔ ISO 7045 H M3 x 12 - 4.8 - H:3
- Mate:770: AASG09 ↔ ISO 7045 H M3 x 12 - 4.8 - H:4
- Mate:771: AASG09 ↔ ISO 7045 H M3 x 12 - 4.8 - H:5
- Mate:772: AASG09 ↔ ISO 7045 H M3 x 12 - 4.8 - H:7
- Mate:773: AASG09 ↔ ISO 7045 H M3 x 12 - 4.8 - H:6
- Mate:774: AASG09 ↔ ISO 7045 H M3 x 12 - 4.8 - H:5
- Mate:775: AASG09 ↔ ISO 7045 H M3 x 12 - 4.8 - H:4
- Mate:776: AASG09 ↔ ISO 7045 H M3 x 12 - 4.8 - H:7
- Mate:777: AASG09 ↔ ISO 7045 H M3 x 12 - 4.8 - H:6
- Mate:778: 12V DC Motor 378-1:3 ↔ ISO 7045 H M3 x 8 - 4.8 - H:5
- Mate:779: 12V DC Motor 378-1:3 ↔ ISO 7045 H M3 x 8 - 4.8 - H:6
- Mate:782: 4mm mounting hub:8 ↔ AASG09
- Mate:783: AA049:1 ↔ Steel Rod 8mm x 80mm:1
- Mate:786: AA049:1 ↔ ISO 4018 M5 x 10:5
- Mate:787: AA049:1 ↔ ISO 4018 M5 x 10:3
- Mate:788: AA049:1 ↔ ISO 4018 M5 x 10:4
- Mate:789: AA049:1 ↔ ISO 4018 M5 x 10:5
- Mate:790: AA049:1 ↔ ISO 4018 M5 x 10:3
- Mate:791: AA049:1 ↔ ISO 4018 M5 x 10:4
- Mate:792: Servo Mounting Hub:1 ↔ ISO 7045 H M3 x 8 - 4.8 - H:9
- Mate:793: Servo Mounting Hub:1 ↔ ISO 7045 H M3 x 8 - 4.8 - H:10
- Mate:794: Servo Mounting Hub:1 ↔ ISO 7045 H M3 x 8 - 4.8 - H:8
- Mate:795: Servo Mounting Hub:1 ↔ ISO 7045 H M3 x 8 - 4.8 - H:7
- Mate:796: Servo Mounting Hub:1 ↔ ISO 7045 H M3 x 8 - 4.8 - H:9
- Mate:797: Servo Mounting Hub:1 ↔ ISO 7045 H M3 x 8 - 4.8 - H:10
- Mate:798: Servo Mounting Hub:1 ↔ ISO 7045 H M3 x 8 - 4.8 - H:8
- Mate:799: Servo Mounting Hub:1 ↔ ISO 7045 H M3 x 8 - 4.8 - H:7
- Mate:800: AA047:1 ↔ ISO 7045 H M3 x 8 - 4.8 - H:11
- Mate:801: AA047:1 ↔ ISO 7045 H M3 x 8 - 4.8 - H:11
- Mate:802: AA006b:1 ↔ ISO 4018 M5 x 25:7
- Mate:803: AA006b:1 ↔ ISO 4018 M5 x 25:7
- Mate:804: AA006b:1 ↔ ISO 4018 M5 x 25:8
- Mate:805: AA006b:1 ↔ ISO 4018 M5 x 25:8
- Mate:806: AA005b:1 ↔ ISO 4018 M5 x 25:9
- Mate:807: AA005b:1 ↔ ISO 4018 M5 x 25:10
- Mate:808: AA005b:1 ↔ ISO 4018 M5 x 25:9
- Mate:809: AA005b:1 ↔ ISO 4018 M5 x 25:10
- Mate:810: AASG01 ↔ ISO 4018 M5 x 25:12
- Mate:811: AASG01 ↔ ISO 4018 M5 x 25:13
- Mate:812: AASG01 ↔ ISO 4018 M5 x 25:11
- Mate:813: AASG01 ↔ ISO 4018 M5 x 25:15
- Mate:814: AASG01 ↔ ISO 4018 M5 x 25:14
- Mate:815: AASG01 ↔ ISO 4018 M5 x 25:16
- Mate:816: AASG01 ↔ ISO 4018 M5 x 25:12
- Mate:817: AASG01 ↔ ISO 4018 M5 x 25:14
- Mate:818: AASG01 ↔ ISO 4018 M5 x 25:16
- Mate:819: AASG01 ↔ ISO 4018 M5 x 25:15
- Mate:820: AASG01 ↔ ISO 4018 M5 x 25:11
- Mate:821: AASG01 ↔ ISO 4018 M5 x 25:13
- Mate:827: AASG05 ↔ ISO 4018 M5 x 25:20
- Mate:828: AASG05 ↔ ISO 4018 M5 x 25:20
- Mate:829: AASG05 ↔ ISO 4018 M5 x 25:18
- Mate:830: AASG05 ↔ ISO 4018 M5 x 25:22
- Mate:831: AASG05 ↔ ISO 4018 M5 x 25:17
- Mate:832: AASG05 ↔ ISO 4018 M5 x 25:19
- Mate:833: AASG05 ↔ ISO 4018 M5 x 25:21
- Mate:838: AA005b:1 ↔ AA006b:1
- Mate:839: AASG02 ↔ ISO 4018 M5 x 25:25
- Mate:841: AASG02 ↔ ISO 4018 M5 x 25:27
- Mate:842: AASG02 ↔ ISO 4018 M5 x 25:28
- Mate:843: AASG02 ↔ ISO 4018 M5 x 25:28
- Mate:844: AASG02 ↔ ISO 4018 M5 x 25:27
- Mate:845: AASG02 ↔ ISO 4018 M5 x 25:25
- Mate:852: ISO 4035 M5:2 ↔ ISO 4018 M5 x 40:2
- Mate:860: AASG03 ↔ ISO 4018 M5 x 25:33
- Mate:861: AASG03 ↔ ISO 4018 M5 x 25:35
- Mate:862: AASG03 ↔ ISO 4018 M5 x 25:34
- Mate:863: AASG03 ↔ ISO 4018 M5 x 25:34
- Mate:864: AASG03 ↔ ISO 4018 M5 x 25:35
- Mate:865: AASG03 ↔ ISO 4018 M5 x 25:33
- Mate:866: AA037:1 ↔ ISO 4018 M5 x 35:1
- Mate:867: AA037:1 ↔ ISO 4018 M5 x 35:1
- Mate:868: AA036:1 ↔ ISO 4018 M5 x 35:2
- Flush:24: ISO 4018 M5 x 35:1 ↔ ISO 4018 M5 x 35:2
- Mate:869: ISO 4035 M5:3 ↔ ISO 4018 M5 x 35:1
- Mate:870: ISO 4035 M5:4 ↔ ISO 4018 M5 x 35:2
- Mate:871: AA036:1 ↔ ISO 4035 M5:4
- Mate:872: AA036:1 ↔ ISO 4035 M5:3
- Mate:873: AA037:1 ↔ ISO 4018 M5 x 25:39
- Mate:874: AA037:1 ↔ ISO 4018 M5 x 25:38
- Mate:875: AA037:1 ↔ ISO 4018 M5 x 25:37
- Mate:876: AA037:1 ↔ ISO 4018 M5 x 25:36
- Flush:25 (-9 mm): AA037:1 ↔ ISO 4018 M5 x 25:39
- Flush:26 (9 mm): AA037:1 ↔ ISO 4018 M5 x 25:38
- Mate:877: AA016b:1 ↔ ISO 4018 M5 x 25:37
- Mate:878: AA016b:1 ↔ ISO 4018 M5 x 25:36
- Mate:879: AA034:1 ↔ ISO 4018 M5 x 25:42
- Mate:880: AA034:1 ↔ ISO 4018 M5 x 25:41
- Mate:881: AA034:1 ↔ ISO 4018 M5 x 25:43
- Mate:882: AA034:1 ↔ ISO 4018 M5 x 25:40
- Mate:883: AA034:1 ↔ ISO 4018 M5 x 25:40
- Mate:884: AA034:1 ↔ ISO 4018 M5 x 25:43
- Mate:885: AA034:1 ↔ ISO 4018 M5 x 25:42
- Mate:886: AA034:1 ↔ ISO 4018 M5 x 25:41
- Mate:887: 4mm mounting hub:1 ↔ AASG01
- Mate:888: AASG01 ↔ ISO 7045 H M3 x 12 - 4.8 - H:9
- Mate:889: AASG01 ↔ ISO 7045 H M3 x 12 - 4.8 - H:8
- Mate:890: AASG01 ↔ ISO 7045 H M3 x 12 - 4.8 - H:8
- Mate:891: AASG01 ↔ ISO 7045 H M3 x 12 - 4.8 - H:9
- Mate:897: AASG02 ↔ ISO 7045 H M3 x 8 - 4.8 - H:13
- Mate:898: AASG02 ↔ ISO 7045 H M3 x 8 - 4.8 - H:14
- Mate:899: AASG02 ↔ ISO 7045 H M3 x 8 - 4.8 - H:15
- Mate:900: AASG02 ↔ ISO 7045 H M3 x 8 - 4.8 - H:13
- Mate:901: AASG02 ↔ ISO 7045 H M3 x 8 - 4.8 - H:14
- Mate:902: AASG02 ↔ ISO 7045 H M3 x 8 - 4.8 - H:15
- Mate:905: AA001c:1 ↔ ISO 4762 M4 x 10:1
- Mate:906: AA001c:1 ↔ ISO 4762 M4 x 10:2
- Mate:907: 12V DC Motor 378-1:6 ↔ ISO 7045 H M3 x 8 - 4.8 - H:17
- Mate:908: 12V DC Motor 378-1:6 ↔ ISO 7045 H M3 x 8 - 4.8 - H:16
- Mate:909: AA005b:1 ↔ ISO 7045 H M3 x 8 - 4.8 - H:17
- Mate:910: AA005b:1 ↔ ISO 7045 H M3 x 8 - 4.8 - H:16
- Mate:911: 8mm Hub:6 ↔ ISO 7045 H M3 x 12 - 4.8 - H:10
- Mate:912: 8mm Hub:6 ↔ ISO 7045 H M3 x 12 - 4.8 - H:12
- Mate:913: 8mm Hub:6 ↔ ISO 7045 H M3 x 12 - 4.8 - H:11
- Mate:914: 8mm Hub:6 ↔ ISO 7045 H M3 x 12 - 4.8 - H:10
- Mate:915: 8mm Hub:6 ↔ ISO 7045 H M3 x 12 - 4.8 - H:11
- Mate:916: 8mm Hub:6 ↔ ISO 7045 H M3 x 12 - 4.8 - H:12
- Mate:917: AASG04 ↔ ISO 7045 H M3 x 12 - 4.8 - H:14
- Mate:918: AASG04 ↔ ISO 7045 H M3 x 12 - 4.8 - H:15
- Mate:919: AASG04 ↔ ISO 7045 H M3 x 12 - 4.8 - H:13
- Mate:920: AASG04 ↔ ISO 7045 H M3 x 12 - 4.8 - H:13
- Mate:921: AASG04 ↔ ISO 7045 H M3 x 12 - 4.8 - H:14
- Mate:922: AASG04 ↔ ISO 7045 H M3 x 12 - 4.8 - H:15
- Mate:939: AA036:1 ↔ ISO 4018 M5 x 25:33
- Mate:948: AA010b:1 ↔ ISO 4762 M4 x 10:4
- Mate:950: AA037:1 ↔ ISO 7045 H M3 x 8 - 4.8 - H:21
- Mate:951: AA037:1 ↔ ISO 7045 H M3 x 8 - 4.8 - H:20
- Mate:952: AA037:1 ↔ ISO 7045 H M3 x 8 - 4.8 - H:21
- Mate:953: AA037:1 ↔ ISO 7045 H M3 x 8 - 4.8 - H:20
- Mate:958: AASG07 ↔ ISO 7045 H M3 x 8 - 4.8 - H:25
- Mate:959: AASG07 ↔ ISO 7045 H M3 x 8 - 4.8 - H:26
- Mate:960: AASG07 ↔ ISO 7045 H M3 x 8 - 4.8 - H:24
- Mate:961: AASG07 ↔ ISO 7045 H M3 x 8 - 4.8 - H:26
- Mate:962: AASG07 ↔ ISO 7045 H M3 x 8 - 4.8 - H:25
- Mate:963: AASG07 ↔ ISO 7045 H M3 x 8 - 4.8 - H:24
- Mate:964: AA034:1 ↔ ISO 7045 H M3 x 8 - 4.8 - H:28
- Mate:965: AA034:1 ↔ ISO 7045 H M3 x 8 - 4.8 - H:27
- Mate:966: AA034:1 ↔ ISO 7045 H M3 x 8 - 4.8 - H:29
- Mate:967: AA034:1 ↔ ISO 7045 H M3 x 8 - 4.8 - H:30
- Mate:968: AA034:1 ↔ ISO 7045 H M3 x 8 - 4.8 - H:32
- Mate:969: AA034:1 ↔ ISO 7045 H M3 x 8 - 4.8 - H:31
- Mate:970: AA034:1 ↔ ISO 7045 H M3 x 8 - 4.8 - H:30
- Mate:971: AA034:1 ↔ ISO 7045 H M3 x 8 - 4.8 - H:29
- Mate:972: AA034:1 ↔ ISO 7045 H M3 x 8 - 4.8 - H:27
- Mate:973: AA034:1 ↔ ISO 7045 H M3 x 8 - 4.8 - H:28
- Mate:974: AA034:1 ↔ ISO 7045 H M3 x 8 - 4.8 - H:32
- Mate:975: AA034:1 ↔ ISO 7045 H M3 x 8 - 4.8 - H:31
- Mate:976: AA014:2 ↔ ISO 4017 M5 x 20:6
- Mate:977: AA014:2 ↔ ISO 4017 M5 x 20:5
- Mate:978: AA014:2 ↔ ISO 4017 M5 x 20:4
- Mate:979: AA014:2 ↔ ISO 4017 M5 x 20:5
- Mate:980: AA014:2 ↔ ISO 4017 M5 x 20:4
- Mate:981: AA014:2 ↔ ISO 4017 M5 x 20:6
- Mate:984: ISO 4035 M5:6 ↔ ISO 4018 M5 x 25:40
- Mate:985: ISO 4035 M5:5 ↔ ISO 4018 M5 x 25:42
- Mate:988: ISO 4035 M5:8 ↔ ISO 4018 M5 x 25:41
- Mate:989: ISO 4035 M5:7 ↔ ISO 4018 M5 x 25:43
- Mate:1027: ISO 4035 M5:10 ↔ ISO 4018 M5 x 40:3
- Mate:1076: AA035c:1 ↔ Steel Rod 8mm x 140mm:1
- Mate:1077: AA035c:1 ↔ AASG02
- Mate:1083: AA001c:1 ↔ TSINY TS-42GZ495:1
- Mate:1084: AA001c:1 ↔ TSINY TS-42GZ495:1
- Mate:1085: AA001c:1 ↔ TSINY TS-42GZ495:1
- Mate:1086: AA001c:1 ↔ TSINY TS-42GZ495:1
- Mate:1088: AA006b:1 ↔ EMS22XXX-D28-LSX:1
- Mate:1089: AA006b:1 ↔ EMS22XXX-D28-LSX:1
- Angle:17 (90 deg): AA006b:1 ↔ EMS22XXX-D28-LSX:1
- Mate:1090: 6mm Mounting Hub:2 ↔ EMS22XXX-D28-LSX:1
- Mate:1091: 6mm Mounting Hub:2 ↔ EMS22XXX-D28-LSX:1
- Mate:1093: AA001c:1 ↔ EMS22XXX-D28-LSX:2
- Angle:18 (180 deg): AA001c:1 ↔ EMS22XXX-D28-LSX:2
- Mate:1095: AA001c:1 ↔ EMS22XXX-D28-LSX:2
- Mate:1097: AA010b:1 ↔ TSINY TS-42GZ495:2
- Mate:1098: AA010b:1 ↔ TSINY TS-42GZ495:2
- Angle:21 (0 deg): AA010b:1 ↔ EMS22XXX-D28-LSX:3
- Mate:1100: AA010b:1 ↔ EMS22XXX-D28-LSX:3
- Mate:1101: AA010b:1 ↔ TSINY TS-42GZ495:2
- Mate:1102: AA010b:1 ↔ TSINY TS-42GZ495:2
- Mate:1104: AA008d2:1 ↔ TSINY TS-42GZ495:3
- Mate:1106: AA008d2:1 ↔ EMS22XXX-D28-LSX:4
- Mate:1107: AA008d2:1 ↔ EMS22XXX-D28-LSX:4
- Angle:22 (0 deg): AA008d2:1 ↔ EMS22XXX-D28-LSX:4
- Mate:1113: AA008c:1 ↔ AA008d2:1
- Mate:1114: AA008c:1 ↔ AA008d2:1
- Mate:1115: AA008c:1 ↔ AA008d2:1
- Mate:1122: AA001c:1 ↔ Steel Rod 8mm x 140mm:1
- Mate:1124: AA008d2:1 ↔ AASG06
- Mate:1125: AA008c:1 ↔ AA008d2:1
- Mate:1126: AA010b:1 ↔ EMS22XXX-D28-LSX:3
- Mate:1128: TSINY TS-42GZ495:2 ↔ AASG03
- Mate:1157: AA008d2:1 ↔ ISO 4018 M5 x 25:29
- Mate:1158: AA008d2:1 ↔ ISO 4018 M5 x 25:32
- Mate:1159: AA008d2:1 ↔ ISO 4018 M5 x 25:29
- Mate:1160: AA008d2:1 ↔ TSINY TS-42GZ495:3
- Mate:1161: AA008d2:1 ↔ TSINY TS-42GZ495:3
- Mate:1162: AA008d2:1 ↔ ISO 4018 M5 x 40:1
- Mate:1163: AA008d2:1 ↔ ISO 4018 M5 x 40:2
- Mate:1164: AA008d2:1 ↔ ISO 4018 M5 x 40:4
- Mate:1165: AA008d2:1 ↔ ISO 4018 M5 x 40:3
- Mate:1166: AA008d2:1 ↔ ISO 4018 M5 x 40:2
- Mate:1167: AA035c:1 ↔ ISO 4035 M5:1
- Mate:1168: AA035c:1 ↔ ISO 4035 M5:1
- Mate:1169: AA035c:1 ↔ ISO 4018 M5 x 40:1
- Mate:1170: AA008d2:1 ↔ AA035c:1
- Mate:1171: AA035c:1 ↔ ISO 4018 M5 x 40:4
- Mate:1172: AA035c:1 ↔ ISO 4018 M5 x 40:3
- Mate:1173: AA035c:1 ↔ ISO 4035 M5:10
- Mate:1174: ISO 4035 M5:9 ↔ ISO 4018 M5 x 40:4
- Mate:1175: AA035c:1 ↔ ISO 4035 M5:9
- Angle:24 (0 deg): AA035c:1 ↔ ISO 4035 M5:9
- Angle:25 (0 deg): AA035c:1 ↔ ISO 4035 M5:10
- Mate:1176: AA035c:1 ↔ ISO 4035 M5:2
- Flush:35: Steel Rod 8mm x 140mm:1 ↔ 8mm Hub:4
- Mate:1177: 6mm Mounting Hub:5 ↔ EMS22XXX-D28-LSX:2
- Mate:1178: 6mm Mounting Hub:5 ↔ AASG04
- Mate:1179: 6mm Mounting Hub:5 ↔ AASG04
- Mate:1180: EMS22XXX-D28-LSX:2 ↔ AASG04
- Mate:1182: EMS22XXX-D28-LSX:1 ↔ AASG05
- Mate:1185: 6mm Mounting Hub:7 ↔ EMS22XXX-D28-LSX:3
- Mate:1186: 6mm Mounting Hub:7 ↔ AASG07
- Mate:1187: EMS22XXX-D28-LSX:3 ↔ AASG07
- Mate:1188: 6mm Mounting Hub:7 ↔ AASG07
- Mate:1190: EMS22XXX-D28-LSX:4 ↔ AASG06
- Mate:1192: AA008d2:1 ↔ ISO 4018 M5 x 25:30
- Mate:1193: AA008d2:1 ↔ ISO 4018 M5 x 25:30
- Mate:1194: AA008d2:1 ↔ ISO 4018 M5 x 25:31
- Mate:1195: AA008d2:1 ↔ ISO 4018 M5 x 25:31
- Mate:1196: AA051:1 ↔ Steel Rod 8mm x 110mm:1
- Mate:1197: AA036:1 ↔ AA051:1
- Mate:1198: AA036:1 ↔ 8mm Hub:14
- Mate:1199: AA036:1 ↔ 8mm Hub:14
- Mate:1200: AA036:1 ↔ 8mm Hub:14
- Mate:1201: AA052:1 ↔ Steel Rod 8mm x 140mm:1
- Mate:1202: AA035c:1 ↔ AA052:1
- Mate:1203: AA035c:1 ↔ 8mm Hub:6
- Mate:1204: AA010b:1 ↔ Steel Rod 8mm x 110mm:1
- Mate:1206: AA016b:1 ↔ EMS22XXX-D28-LSX:5
- Mate:1207: AA016b:1 ↔ EMS22XXX-D28-LSX:5
- Angle:26 (180 deg): AA016b:1 ↔ EMS22XXX-D28-LSX:5
- Mate:1210: EMS22XXX-D28-LSX:5 ↔ 6mm Mounting Hub, thin:2
- Mate:1211: AA045b:1 ↔ EMS22XXX-D28-LSX:6
- Mate:1212: AA045b:1 ↔ EMS22XXX-D28-LSX:6
- Angle:27 (0 deg): AA045b:1 ↔ EMS22XXX-D28-LSX:6
- Mate:1213: AA034:1 ↔ AA045b:1
- Mate:1214: AA045b:1 ↔ ISO 4018 M5 x 25:41
- Mate:1215: AA045b:1 ↔ ISO 4018 M5 x 25:43
- Mate:1216: AA045b:1 ↔ Steel Rod 8mm x 80mm:1
- Mate:1217 (1 mm): AA045b:1 ↔ AA046:1
- Mate:1218: AA045b:1 ↔ AA049:1
- Mate:1219: AA045b:1 ↔ ISO 4018 M5 x 10:5
- Flush:37 (-2.5 mm): AA045b:1 ↔ Steel Rod 8mm x 80mm:1
- Mate:1221: AA045b:1 ↔ AASG10
- Mate:1223: AA045b:1 ↔ AASG09
- Mate:1224: AA045b:1 ↔ 12V DC Motor 378-1:3
- Mate:1225: AA045b:1 ↔ 12V DC Motor 378-1:3
- Mate:1226: 4mm mounting hub:8 ↔ AASG09
- Mate:1227: AA045b:1 ↔ AASG09
- Mate:1228: 6mm Mounting Hub:10 ↔ EMS22XXX-D28-LSX:6
- Mate:1230: QS12MM250:1 ↔ AASG05
- Mate:1232: EMS22XXX-D28-LSX:1 ↔ AASG05
- Mate:1233: AA006b:1 ↔ AASG05
- Mate:1234: Steel Rod 8mm x 80mm:1 ↔ 8mm Hub:8
- Mate:1235: AA045b:1 ↔ AASG10
- Mate:1256: AA034:1 ↔ ISO 7045 H M3 x 8 - 4.8 - H:30
- Mate:1258: AA010b:1 ↔ AA053:1
- Mate:1259: AA010b:1 ↔ AA053:1
- Mate:1260 (0.5 mm): AA010b:1 ↔ AA053:1
- Mate:1261: AA001c:1 ↔ AA053:3
- Mate:1262: AA001c:1 ↔ AA053:3
- Mate:1263 (0.5 mm): AA001c:1 ↔ AA053:3
- Mate:1264: AA045b:1 ↔ 22x8x8mm Bearing:6
- Mate:1265: AA045b:1 ↔ 22x8x8mm Bearing:5
- Mate:1267: EMS22XXX-D28-LSX:6 ↔ AASG10
- Mate:1268: AASG06 ↔ ISO 7045 H M3 x 12 - 4.8 - H:32
- Mate:1269: AASG06 ↔ ISO 7045 H M3 x 12 - 4.8 - H:32
- Mate:1270: AA054:1 ↔ TSINY TS-42GZ495:3
- Mate:1271: AA054:1 ↔ TSINY TS-42GZ495:3
- Mate:1274: AA010b:1 ↔ AA055:1
- Mate:1275: AA054:1 ↔ AA055:1
- Mate:1276: AA010b:1 ↔ AA054:1
- Mate:1277: AA010b:1 ↔ AA055:1
- Mate:1278: AA001c:1 ↔ AA004:1
- Mate:1279: AA001c:1 ↔ AASG01
- Mate:1280: AA001c:1 ↔ AASG01
- Mate:1281: AA013:2 ↔ ISO 4017 M5 x 20:1
- Mate:1282: AA054:1 ↔ AASG06
- Mate:1283: Steel Rod 8mm x 110mm:1 ↔ 6mm Mounting Hub:11
- Mate:1284: 6mm Mounting Hub:11 ↔ AASG07
- Mate:1290: 12V DC Motor 378-1:4 ↔ AS 1421 Flat Point - Metric M4 x 10 Flat Point:2
- Mate:1292: 12V DC Motor 378-1:4 ↔ 6mm x 120mm D Shaft:1
- Mate:1293: AA057:1 ↔ TSINY TS-42GZ495:1
- Angle:1295 (180 deg): AA057:1 ↔ TSINY TS-42GZ495:1
- Mate:1294: AA001c:1 ↔ AA057:1
- Mate:1295: AA057:1 ↔ AASG02
- Mate:1296: AA046:1 ↔ AASG09
- Mate:1297: AA046:1 ↔ AASG09
- Mate:1298: Steel Rod 8mm x 80mm:1 ↔ 8mm Hub:9
- Mate:1299: Steel Rod 8mm x 80mm:1 ↔ 8mm Hub:9
- Mate:1300: AA057:2 ↔ TSINY TS-42GZ495:2
- Angle:1296 (180 deg): AA057:2 ↔ TSINY TS-42GZ495:2
- Mate:1301: AA010b:1 ↔ AA057:2
- Mate:1302: AA057:2 ↔ AASG03
- Mate:1303: 12V DC Motor 378-1:4 ↔ 6mm x 120mm D Shaft:1
- Mate:1304: 12V DC Motor 378-1:4 ↔ 6mm x 120mm D Shaft:1
- Mate:1305: 6mm x 120mm D Shaft:1 ↔ AASG08
- Mate:1306: 8mm Hub:2 ↔ 6mm x 120mm D Shaft:1
- Mate:1308: 22x8x8mm Bearing:7 ↔ 6mm x 120mm D Shaft:1
- Mate:1309: AA034:1 ↔ 6mm x 120mm D Shaft:1
- Mate:1310: AA034:1 ↔ AA045b:1
- Mate:1311: AA034:1 ↔ AA045b:1
- Angle:1297 (0 deg): AA035c:1 ↔ TSINY TS-42GZ495:3
- Mate:1312: AA008d2:1 ↔ AA035c:1
- Mate:1313: EMS22XXX-D28-LSX:4 ↔ 6mm Mounting Hub, thin:1
- Mate:1314: AASG06 ↔ 6mm Mounting Hub, thin:1
- Mate:1315: AASG06 ↔ 6mm Mounting Hub, thin:1
- Mate:1316: EMS22XXX-D28-LSX:5 ↔ 6mm Mounting Hub, thin:2
- Mate:1317: AASG08 ↔ 6mm Mounting Hub, thin:2
- Mate:1318: 6mm x 120mm D Shaft:1 ↔ 6mm Mounting Hub, thin:3
- Mate:1319: AASG08 ↔ 6mm Mounting Hub, thin:3
- Mate:1320: AA054:1 ↔ 8mm Mounting Hub, thin:1
- Mate:1321: AASG06 ↔ 8mm Mounting Hub, thin:1
- Mate:1322: AASG06 ↔ 8mm Mounting Hub, thin:1
- Mate:1323: 6mm Mounting Hub:10 ↔ AASG10
- Mate:1324: 8mm Hub:8 ↔ AASG10
- Mate:1325: 8mm Hub:8 ↔ AASG10
- Mate:1326: EMS22XXX-D28-LSX:5 ↔ AASG08
